# Autodesk Inventor assembly: catapfc4
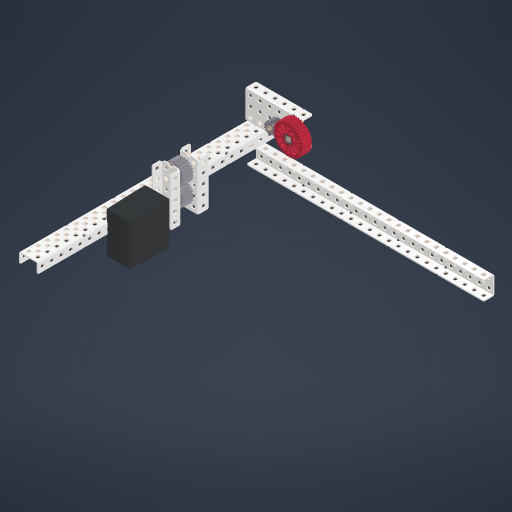
[picture p0: Inventor's stored thumbnail of the model, 512x512]
Saved by Autodesk Inventor 2024 (Build 280153000, 153)
## iProperties
Created: 2023-10-21
Part Number: catapfc4
Document SubType Name: Assembly
Designer: macbook
Author: macbook
## Documents named in this file (9)
- \\Mac\Home\Desktop\code\1599V-VRC\Cad\Assembly\v2\catapfc4.iam
- \\Mac\Home\Desktop\code\1599V-VRC\Cad\Structure\C Channel\Aluminum 1x2x1\Alu C 1x2x1x25.ipt
- \\Mac\Home\Desktop\code\1599V-VRC\Cad\Electronics\V5 Simple Motor.ipt
- \\Mac\Home\Desktop\code\1599V-VRC\Cad\Motion\Gears\HS Gear\HS 12T Gear, No Insert.iam
- \\Mac\Home\Desktop\code\1599V-VRC\Cad\Motion\Gears\HS Gear.iam
- \\Mac\Home\Desktop\code\1599V-VRC\Cad\Motion\Gears\HS Gear\HS 24T Gear, No Insert.iam
- \\Mac\Home\Desktop\code\1599V-VRC\Cad\Motion\Gears\HS Gear\HS 36T Gear, No Insert.iam
- \\Mac\Home\Desktop\code\1599V-VRC\Cad\Structure\C Channel\Aluminum 1x3x1\Alu C 1x3x1x6.ipt
- \\Mac\Home\Desktop\code\1599V-VRC\Cad\Structure\C Channel\Aluminum 1x2x1\Alu C 1x2x1x5.ipt
## Components (10 placed, 7 different names)
1. Alu C 1x2x1x25:1
2. Alu C 1x2x1x25:2 — Insert:7, Insert:10, Insert:14
3. V5 Simple Motor:1 — Insert:15
4. HS 12T Gear, No Insert:1 [sub-assembly] — Insert:9
5. HS 24T Gear, No Insert:2 [sub-assembly] — Insert:13
6. HS 24T Gear, No Insert:4 [sub-assembly] — Insert:12
7. HS 36T Gear, No Insert:6 [sub-assembly] — Insert:8
8. Alu C 1x3x1x6:3 — Insert:7, Insert:8, Insert:9
9. Alu C 1x2x1x5:1 — Insert:10, Insert:12, Insert:13
10. Alu C 1x2x1x5:3 — Insert:14, Insert:15
## Relationships (10: Insert 10)
- [Insert] (25.4 mm): Alu C 1x2x1x25:1 ↔ Alu C 1x2x1x25:2
- [Insert] (25.4 mm): Alu C 1x2x1x25:1 ↔ Alu C 1x2x1x25:2
- Insert:7: Alu C 1x2x1x25:2 ↔ Alu C 1x3x1x6:3
- Insert:8: HS 36T Gear, No Insert:6 ↔ Alu C 1x3x1x6:3
- Insert:9: HS 12T Gear, No Insert:1 ↔ Alu C 1x3x1x6:3
- Insert:10: Alu C 1x2x1x25:2 ↔ Alu C 1x2x1x5:1
- Insert:12 (6.35 mm): HS 24T Gear, No Insert:4 ↔ Alu C 1x2x1x5:1
- Insert:13 (6.35 mm): HS 24T Gear, No Insert:2 ↔ Alu C 1x2x1x5:1
- Insert:14: Alu C 1x2x1x25:2 ↔ Alu C 1x2x1x5:3
- Insert:15: V5 Simple Motor:1 ↔ Alu C 1x2x1x5:3
